# Autodesk Inventor assembly: Assembly_Matchboxscope_injectionmolded_holo
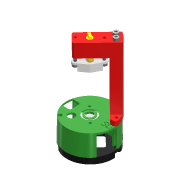
[picture p0: Inventor's stored thumbnail of the model, 180x180]
Saved by Autodesk Inventor 2022 (Build 260153000, 153)
## iProperties
Created: 2023-04-12
Part Number: Assembly_Matchboxscope_injectionmolded_holo
Document SubType Name: Assembly
Designer: diederichbenedict
Author: diederichbenedict
## Documents named in this file (10)
- C:\Users\diederichbenedict\Dropbox\Dokumente\Promotion\PROJECTS\Matchboxscope\INVENTOR\RELEASE\InjectionMolded\Assembly_Matchboxscope_injectionmolded_holo.iam
- C:\Users\diederichbenedict\Dropbox\Dokumente\Promotion\PROJECTS\Matchboxscope\INVENTOR\RELEASE\InjectionMolded\IM_Matchboxscope_base.ipt
- C:\Users\diederichbenedict\Dropbox\Dokumente\Promotion\PROJECTS\Matchboxscope\INVENTOR\RELEASE\InjectionMolded\IM_Matchboxscope_plate.ipt
- C:\Users\diederichbenedict\Dropbox\Dokumente\Promotion\PROJECTS\Matchboxscope\INVENTOR\RELEASE\InjectionMolded\Anglerfish_Cameraspacer.ipt
- C:\Users\diederichbenedict\Dropbox\Dokumente\Promotion\PROJECTS\Matchboxscope\INVENTOR\RELEASE\InjectionMolded\00_laserpointer_red.ipt
- C:\Users\diederichbenedict\Dropbox\Dokumente\Promotion\PROJECTS\Matchboxscope\INVENTOR\RELEASE\InjectionMolded\00_mk8_nozzle_0.4STEP.ipt
- C:\Users\diederichbenedict\Dropbox\Dokumente\Promotion\PROJECTS\Matchboxscope\INVENTOR\RELEASE\InjectionMolded\IM_Matchboxscope_Laserholder.ipt
- C:\Users\diederichbenedict\Dropbox\Dokumente\Promotion\PROJECTS\Matchboxscope\INVENTOR\RELEASE\InjectionMolded\IM_Matchboxscope_Laserholder_2.ipt
- C:\Users\diederichbenedict\Dropbox\Dokumente\Promotion\PROJECTS\Matchboxscope\INVENTOR\RELEASE\InjectionMolded\IM_Lensholder.ipt
- C:\Users\diederichbenedict\Documents\Inventor\Content Center Files\R2022\de-DE\DIN 912\DIN 912 - M3 x 0.5 x 16 x 14.75.ipt
## Components (13 placed, 9 different names)
1. IM_Matchboxscope_base:1 — Passend:1, Passend:2, Fluchtend:1, Fluchtend:2
2. IM_Matchboxscope_plate:1 — Einfügen:9
3. Anglerfish_Cameraspacer:1
4. 00_laserpointer_red:2 — Einfügen:3, Passend:1
5. 00_mk8_nozzle_0.4STEP:1 — Einfügen:3, Passend:2
6. IM_Matchboxscope_Laserholder:1 — Fluchtend:1, Fluchtend:2, Fluchtend:3
7. IM_Matchboxscope_Laserholder_2:1 — Fluchtend:3, Einfügen:4, Einfügen:5, Einfügen:6
8. IM_Lensholder:1 — Einfügen:4, Einfügen:7, Einfügen:8
9. DIN 912 - ersetzt durch DIN EN ISO 4762 M3 x 16:1 — Einfügen:5
10. DIN 912 - ersetzt durch DIN EN ISO 4762 M3 x 16:2 — Einfügen:6
11. DIN 912 - ersetzt durch DIN EN ISO 4762 M3 x 16:3 — Einfügen:7
12. DIN 912 - ersetzt durch DIN EN ISO 4762 M3 x 16:4 — Einfügen:8
13. DIN 912 - ersetzt durch DIN EN ISO 4762 M3 x 16:5 — Einfügen:9
## Relationships (14: Insert 9, Flush 3, Mate 2)
- [Insert]: IM_Matchboxscope_base:1 ↔ IM_Matchboxscope_plate:1
- [Insert]: IM_Matchboxscope_base:1 ↔ IM_Matchboxscope_plate:1
- Einfügen:3 [Insert] (2 mm): 00_laserpointer_red:2 ↔ 00_mk8_nozzle_0.4STEP:1
- Passend:1 [Mate]: IM_Matchboxscope_base:1 ↔ 00_laserpointer_red:2
- Passend:2 [Mate] (50 mm): IM_Matchboxscope_base:1 ↔ 00_mk8_nozzle_0.4STEP:1
- Fluchtend:1 [Flush]: IM_Matchboxscope_base:1 ↔ IM_Matchboxscope_Laserholder:1
- Fluchtend:2 [Flush]: IM_Matchboxscope_base:1 ↔ IM_Matchboxscope_Laserholder:1
- Fluchtend:3 [Flush]: IM_Matchboxscope_Laserholder:1 ↔ IM_Matchboxscope_Laserholder_2:1
- Einfügen:4 [Insert] (7 mm): IM_Matchboxscope_Laserholder_2:1 ↔ IM_Lensholder:1
- Einfügen:5 [Insert]: IM_Matchboxscope_Laserholder_2:1 ↔ DIN 912 - ersetzt durch DIN EN ISO 4762 M3 x 16:1
- Einfügen:6 [Insert]: IM_Matchboxscope_Laserholder_2:1 ↔ DIN 912 - ersetzt durch DIN EN ISO 4762 M3 x 16:2
- Einfügen:7 [Insert]: IM_Lensholder:1 ↔ DIN 912 - ersetzt durch DIN EN ISO 4762 M3 x 16:3
- Einfügen:8 [Insert]: IM_Lensholder:1 ↔ DIN 912 - ersetzt durch DIN EN ISO 4762 M3 x 16:4
- Einfügen:9 [Insert] (5 mm): IM_Matchboxscope_plate:1 ↔ DIN 912 - ersetzt durch DIN EN ISO 4762 M3 x 16:5
